# Autodesk Inventor assembly: Assembly1
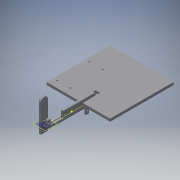
[picture p0: Inventor's stored thumbnail of the model, 180x180]
Saved by Autodesk Inventor 2018 (Build 220112000, 112)
## iProperties
Created: 2018-09-19
Part Number: Assembly1
Document SubType Name: Assembly
Designer: Viraj Shah
Author: Viraj Shah
## Documents named in this file (5)
- C:\Users\Viraj Shah\Documents\Inventor\Crawler\Assembly1.iam
- C:\Users\Viraj Shah\Documents\Inventor\Crawler\Arm1.ipt
- C:\Users\Viraj Shah\Documents\Inventor\Crawler\Arm2.ipt
- C:\Users\Viraj Shah\Documents\Inventor\Crawler\MainBoard.ipt
- C:\Users\Viraj Shah\Documents\Inventor\Crawler\RPI_Zero.ipt
## Components (4 placed, 4 different names)
1. Arm1:2 — Flush:1, Flush:2, Mate:1, Rotational:1
2. Arm2:2 — Mate:1, Rotational:1
3. MainBoard:1 — Flush:1, Flush:2, Mate:2, Mate:3, Flush:3
4. RPI_Zero:1 — Mate:2, Mate:3, Flush:3
## Relationships (7: Flush 3, Mate 3, RevoluteJoint 1)
- Flush:1: Arm1:2 ↔ MainBoard:1
- Flush:2 (-6.5 mm): Arm1:2 ↔ MainBoard:1
- Mate:1 (5 mm): Arm1:2 ↔ Arm2:2
- Rotational:1 [RevoluteJoint] (-5 mm): Arm1:2 ↔ Arm2:2
- Mate:2: MainBoard:1 ↔ RPI_Zero:1
- Mate:3 (-15 mm): MainBoard:1 ↔ RPI_Zero:1
- Flush:3 (10 mm): MainBoard:1 ↔ RPI_Zero:1
